# Autodesk Inventor assembly: rope_pulley_MIR
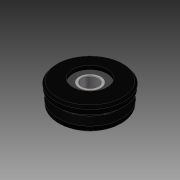
[picture p0: Inventor's stored thumbnail of the model, 180x180]
Saved by Autodesk Inventor 2014 (Build 180170000, 170)
## iProperties
Created: 2014-04-04
Part Number: rope_pulley_MIR
Document SubType Name: Assembly
Designer: buben
Author: buben
## Documents named in this file (3)
- C:\Users\buben\Documents\GitHub\bacon\inventor files\utils\rope_pulley_MIR.iam
- C:\Users\buben\Documents\GitHub\bacon\inventor files\3rd party components\bearing_608\Imported Components\608RS\608RS_MIR.ipt
- C:\Users\buben\Documents\GitHub\bacon\inventor files\utils\rope_pulley_MIR.ipt
## Components (3 placed, 2 different names)
1. 608RS_MIR:1 — Mate:2, Mate:1, Mate:4, Mate:3, Mate:7
2. rope_pulley_MIR:1 — Mate:4, Mate:3, Mate:6, Mate:5
3. rope_pulley_MIR:2 — Mate:7, Mate:6, Mate:5
## Relationships (7: Mate 7)
- Mate:2: 608RS_MIR:1
- Mate:1: 608RS_MIR:1
- Mate:4: 608RS_MIR:1 ↔ rope_pulley_MIR:1
- Mate:3: 608RS_MIR:1 ↔ rope_pulley_MIR:1
- Mate:7: 608RS_MIR:1 ↔ rope_pulley_MIR:2
- Mate:6: rope_pulley_MIR:1 ↔ rope_pulley_MIR:2
- Mate:5: rope_pulley_MIR:1 ↔ rope_pulley_MIR:2
